# Autodesk Inventor assembly: Evaporator
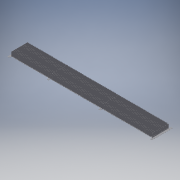
[picture p0: Inventor's stored thumbnail of the model, 180x180]
Saved by Autodesk Inventor 2016 (Build 200138000, 138)
## iProperties
Created: 2017-06-28
Part Number: Evaporator
Document SubType Name: Assembly
Designer: Roeder
Author: Roeder
## Documents named in this file (4)
- T:\07 Projects\2017\Gen3 Indis\01_Documents\Evaporator Specification\Model\Evaporator.iam
- T:\07 Projects\2017\Gen3 Indis\01_Documents\Evaporator Specification\Model\Parts\Baseplate.ipt
- T:\07 Projects\2017\Gen3 Indis\01_Documents\Evaporator Specification\Model\Parts\Cover Plate.ipt
- T:\07 Projects\2017\Gen3 Indis\01_Documents\Evaporator Specification\Model\Parts\Fin.ipt
## Components (6 placed, 3 different names)
1. Baseplate:1 — Flush:1, Flush:2, Rigid:1, Rigid:2, Rigid:3, Flush:3, Flush:4
2. Cover Plate:1 — Flush:1, Flush:2
3. Cover Plate:2 — Rigid:1
4. Cover Plate:3 — Rigid:2
5. Cover Plate:4 — Rigid:3
6. Fin:1 — Flush:3, Flush:4
## Relationships (7: Flush 4, WeldJoint 3)
- Flush:1: Baseplate:1 ↔ Cover Plate:1
- Flush:2: Baseplate:1 ↔ Cover Plate:1
- Rigid:1 [WeldJoint]: Baseplate:1 ↔ Cover Plate:2
- Rigid:2 [WeldJoint]: Baseplate:1 ↔ Cover Plate:3
- Rigid:3 [WeldJoint]: Baseplate:1 ↔ Cover Plate:4
- Flush:3: Baseplate:1 ↔ Fin:1
- Flush:4: Baseplate:1 ↔ Fin:1
